# Autodesk Inventor assembly: Assembly1
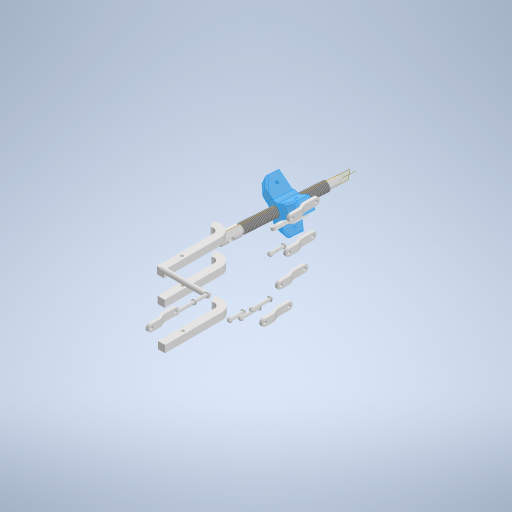
[picture p0: Inventor's stored thumbnail of the model, 512x512]
Saved by Autodesk Inventor 2024.2 (Build 282272000, 272)
## iProperties
Created: 2024-03-04
Part Number: Assembly1
Document SubType Name: Assembly
Designer: 082220042
Author: 082220042
## Documents named in this file (8)
- Z:\EC_Engenharia_da_computacao\desenho_digital\atividade\atividade_14A\Assembly1.iam
- Z:\EC_Engenharia_da_computacao\desenho_digital\atividade\atividade_14A\atividade_14A.ipt
- Z:\EC_Engenharia_da_computacao\desenho_digital\atividade\atividade_14A\atividade_14A_eixo.ipt
- Z:\EC_Engenharia_da_computacao\desenho_digital\atividade\atividade_14A\atividade_14A_garra.ipt
- Z:\EC_Engenharia_da_computacao\desenho_digital\atividade\atividade_14A\atividade_14A_pino_superior.ipt
- Z:\EC_Engenharia_da_computacao\desenho_digital\atividade\atividade_14A\atividade_14A_pino27.ipt
- Z:\EC_Engenharia_da_computacao\desenho_digital\atividade\atividade_14A\atividade_14A_pino37.ipt
- Z:\EC_Engenharia_da_computacao\desenho_digital\atividade\atividade_14A\atividade_14A_uniao.ipt
## Components (18 placed, 7 different names)
1. atividade_14A:1 — Cylindrical:1, Mate:1, Mate:2
2. atividade_14A_eixo:1 — Cylindrical:1
3. atividade_14A_garra:1
4. atividade_14A_pino_superior:1
5. atividade_14A_pino27:1
6. atividade_14A_pino37:1
7. atividade_14A_uniao:1
8. atividade_14A_garra:2
9. atividade_14A_garra:3
10. atividade_14A_pino27:2
11. atividade_14A_pino27:3
12. atividade_14A_pino37:2
13. atividade_14A_pino37:3
14. atividade_14A_uniao:2 — Mate:1, Mate:2
15. atividade_14A_uniao:3
16. atividade_14A_uniao:4
17. atividade_14A_uniao:5
18. atividade_14A_uniao:6
## Relationships (3: Mate 2, CylindricalJoint 1)
- Cylindrical:1: atividade_14A:1 ↔ atividade_14A_eixo:1
- Mate:1: atividade_14A:1 ↔ atividade_14A_uniao:2
- Mate:2: atividade_14A:1 ↔ atividade_14A_uniao:2
